# Autodesk Inventor assembly: chassis weldment
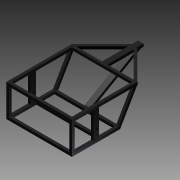
[picture p0: Inventor's stored thumbnail of the model, 180x180]
Saved by Autodesk Inventor 2012 (Build 160160000, 160)
## iProperties
Created: 2011-09-30
Part Number: chassis weldment
Document SubType Name: Weldment
Designer: Antonella
Weld Material: Welded Aluminum-6061
Author: Antonella
## Documents named in this file (3)
- C:\Users\Antonella\Documents\GCC Robotics 2012 - Mechanical\Robot 2.0\Chassis\chassis weldment.iam
- C:\Users\Antonella\Documents\GCC Robotics 2012 - Mechanical\Robot 2.0\Chassis\chassis weldment bottom.iam
- C:\Users\Antonella\Documents\GCC Robotics 2012 - Mechanical\Robot 2.0\Chassis\chassis weldment top.iam
## Components (2 placed, 2 different names)
1. chassis weldment top:1 [sub-assembly] — Mate:5, Flush:3, Flush:4
2. chassis weldment bottom:1 [sub-assembly] — Mate:5, Flush:3, Flush:4
## Relationships (3: Flush 2, Mate 1)
- Mate:5: chassis weldment top:1 ↔ chassis weldment bottom:1
- Flush:3: chassis weldment top:1 ↔ chassis weldment bottom:1
- Flush:4: chassis weldment top:1 ↔ chassis weldment bottom:1
